# Autodesk Inventor assembly: mould_base_p1
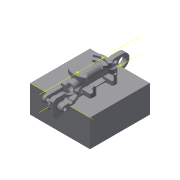
[picture p0: Inventor's stored thumbnail of the model, 180x180]
Saved by Autodesk Inventor 2017 (Build 210142000, 142)
## iProperties
Created: 2018-06-07
Part Number: mould_base_p1
Document SubType Name: Assembly
Designer: Nic
Author: Nic
## Documents named in this file (3)
- C:\Users\Nic\Documents\Antenna\mould_base_p1.iam
- C:\Users\Nic\Documents\Antenna\mould_casing.ipt
- C:\Users\Nic\Documents\Antenna\middle_segment_v2.ipt
## Components (2 placed, 2 different names)
1. mould_casing:1 — Mate:1, Mate:2, Flush:1, Cylindrical:1, Mate:3, Mate:4, Mate:5, Mate:6, Mate:7
2. middle_segment_v2:1 — Flush:1, Cylindrical:1, Mate:8
## Relationships (10: Mate 8, Flush 1, CylindricalJoint 1)
- Mate:1: mould_casing:1
- Mate:2: mould_casing:1
- Flush:1: mould_casing:1 ↔ middle_segment_v2:1
- Cylindrical:1: mould_casing:1 ↔ middle_segment_v2:1
- Mate:3: mould_casing:1
- Mate:4: mould_casing:1
- Mate:5: mould_casing:1
- Mate:6: mould_casing:1
- Mate:7: mould_casing:1
- Mate:8: middle_segment_v2:1
